# Autodesk Inventor assembly: HingeSubassembly
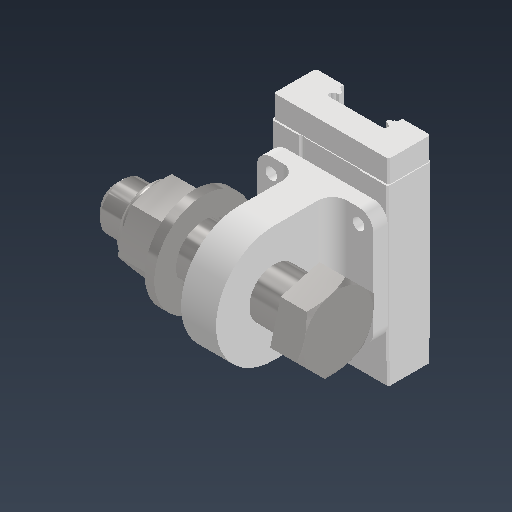
[picture p0: Inventor's stored thumbnail of the model, 512x512]
Saved by Autodesk Inventor 2021 (Build 250183000, 183)
## iProperties
Created: 2021-01-30
Part Number: HingeSubassembly
Document SubType Name: Assembly
Designer: argon
Author: argon
## Documents named in this file (6)
- C:\Users\argon\OneDrive\Documents\GrabCAD\EngOne Maroons\Table Subassemly\HingeSubassembly.iam
- C:\Users\argon\OneDrive\Documents\GrabCAD\EngOne Maroons\Table Subassemly\Table Post\Hinge.ipt
- C:\Users\argon\OneDrive\Documents\GrabCAD\EngOne Maroons\Table Subassemly\Table Post\Ball Bearing Carriage.ipt
- C:\Users\argon\OneDrive\Documents\GrabCAD\EngOne Maroons\McMaster-Carr Parts\97713A129_NO THREADS_ METRIC STEEL HEX HEAD SHOULDER SCREWS.ipt
- C:\Users\argon\OneDrive\Documents\GrabCAD\EngOne Maroons\McMaster-Carr Parts\94645A250_NO THREADS_HIGH-STRENGTH STEEL NYLON-INSERT LOCKNUT.ipt
- C:\Users\argon\OneDrive\Documents\GrabCAD\EngOne Maroons\McMaster-Carr Parts\93475A315_TYPE 18-8 STAINLESS STEEL FLAT WASHER.ipt
## Components (5 placed, 5 different names)
1. Hinge:1 — Mate:1, Mate:2, Mate:3, Mate:4, Mate:9
2. Ball Bearing Carriage:1 — Mate:1, Mate:2, Mate:3
3. 97713A129_NO THREADS_ METRIC STEEL HEX HEAD SHOULDER SCREWS:1 — Mate:4, Mate:5, Mate:6, Mate:7, Mate:9
4. 94645A250_NO THREADS_HIGH-STRENGTH STEEL NYLON-INSERT LOCKNUT:1 — Mate:5, Mate:6, Mate:8
5. 93475A315_TYPE 18-8 STAINLESS STEEL FLAT WASHER:1 — Mate:7, Mate:8
## Relationships (9: Mate 9)
- Mate:1: Hinge:1 ↔ Ball Bearing Carriage:1
- Mate:2: Hinge:1 ↔ Ball Bearing Carriage:1
- Mate:3: Hinge:1 ↔ Ball Bearing Carriage:1
- Mate:4: Hinge:1 ↔ 97713A129_NO THREADS_ METRIC STEEL HEX HEAD SHOULDER SCREWS:1
- Mate:5: 97713A129_NO THREADS_ METRIC STEEL HEX HEAD SHOULDER SCREWS:1 ↔ 94645A250_NO THREADS_HIGH-STRENGTH STEEL NYLON-INSERT LOCKNUT:1
- Mate:6: 97713A129_NO THREADS_ METRIC STEEL HEX HEAD SHOULDER SCREWS:1 ↔ 94645A250_NO THREADS_HIGH-STRENGTH STEEL NYLON-INSERT LOCKNUT:1
- Mate:7: 97713A129_NO THREADS_ METRIC STEEL HEX HEAD SHOULDER SCREWS:1 ↔ 93475A315_TYPE 18-8 STAINLESS STEEL FLAT WASHER:1
- Mate:8: 94645A250_NO THREADS_HIGH-STRENGTH STEEL NYLON-INSERT LOCKNUT:1 ↔ 93475A315_TYPE 18-8 STAINLESS STEEL FLAT WASHER:1
- Mate:9 (12 mm): Hinge:1 ↔ 97713A129_NO THREADS_ METRIC STEEL HEX HEAD SHOULDER SCREWS:1
